# Autodesk Inventor assembly: Membran_Platte_V4_1
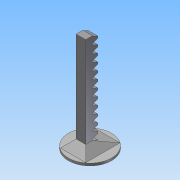
[picture p0: Inventor's stored thumbnail of the model, 180x180]
Saved by Autodesk Inventor 2015 (Build 190159000, 159)
## iProperties
Created: 2015-09-10
Part Number: Membran_Platte_V4_1
Document SubType Name: Assembly
Designer: Johann
Author: Johann
## Documents named in this file (3)
- C:\Users\Johann\Documents\Uni\Bachelorarbeit\Inventor\Membran_Platte_V4_1.iam
- C:\Users\Johann\Documents\Uni\Bachelorarbeit\Inventor\Membran_Platte_V4.ipt
- C:\Users\Johann\Documents\Uni\Bachelorarbeit\Inventor\Zahnstange.ipt
## Components (2 placed, 2 different names)
1. Membran_Platte_V4:1 — Passend:1, Fluchtend:1, Fluchtend:2, Fluchtend:3, Passend:2, Passend:3
2. Zahnstange:1 — Passend:1, Passend:2, Passend:3, Fluchtend:4
## Relationships (7: Flush 4, Mate 3)
- Passend:1 [Mate]: Membran_Platte_V4:1 ↔ Zahnstange:1
- Fluchtend:1 [Flush]: Membran_Platte_V4:1
- Fluchtend:2 [Flush]: Membran_Platte_V4:1
- Fluchtend:3 [Flush]: Membran_Platte_V4:1
- Passend:2 [Mate]: Membran_Platte_V4:1 ↔ Zahnstange:1
- Passend:3 [Mate]: Membran_Platte_V4:1 ↔ Zahnstange:1
- Fluchtend:4 [Flush]: Zahnstange:1
